# Autodesk Inventor assembly: Baugruppe_Montage_Ring_Vorne
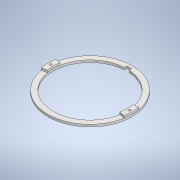
[picture p0: Inventor's stored thumbnail of the model, 180x180]
Saved by Autodesk Inventor 2022.2 (Build 262287010, 287A)
## iProperties
Created: 2024-01-10
Part Number: Baugruppe_Montage_Ring_Vorne
Document SubType Name: Assembly
Designer: ppovolni
Author: ppovolni
## Documents named in this file (4)
- D:\3_Local_Projekte\Weitere_Projekte\weitere_hw_projekte\Hallmesssonde - 8fach_Hallsensor\6_Entwurf Zylinderspule für Kalibrierung\Zylinderspule_Kalibrierung\CAD_Zylinderspule\Baugruppe_Montage_Ring_Vorne.iam
- D:\3_Local_Projekte\Weitere_Projekte\weitere_hw_projekte\Hallmesssonde - 8fach_Hallsensor\6_Entwurf Zylinderspule für Kalibrierung\Zylinderspule_Kalibrierung\CAD_Zylinderspule\Montage_Ring_Vorne.ipt
- D:\3_Local_Projekte\Weitere_Projekte\weitere_hw_projekte\Hallmesssonde - 8fach_Hallsensor\6_Entwurf Zylinderspule für Kalibrierung\Zylinderspule_Kalibrierung\CAD_Zylinderspule\Montage_Ring_Vorne_Aufdickung_Gewinde.ipt
- D:\3_Local_Projekte\Weitere_Projekte\weitere_hw_projekte\Hallmesssonde - 8fach_Hallsensor\6_Entwurf Zylinderspule für Kalibrierung\Zylinderspule_Kalibrierung\CAD_Zylinderspule\Montage_Ring_Vorne_Aufdickung_Gewinde_MIR.ipt
## Components (3 placed, 3 different names)
1. Montage_Ring_Vorne:1 — Fluchtend:1, Fluchtend:2
2. Montage_Ring_Vorne_Aufdickung_Gewinde:1 — Fluchtend:1, Fluchtend:2
3. Montage_Ring_Vorne_Aufdickung_Gewinde_MIR:1
## Relationships (2: Flush 2)
- Fluchtend:1 [Flush]: Montage_Ring_Vorne:1 ↔ Montage_Ring_Vorne_Aufdickung_Gewinde:1
- Fluchtend:2 [Flush]: Montage_Ring_Vorne:1 ↔ Montage_Ring_Vorne_Aufdickung_Gewinde:1
